# Autodesk Inventor assembly: 3 dubbele lagerblok assemble
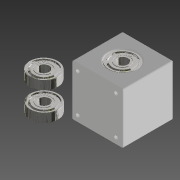
[picture p0: Inventor's stored thumbnail of the model, 180x180]
Saved by Autodesk Inventor 2020 (Build 240168000, 168)
## iProperties
Created: 2020-05-19
Part Number: 3 dubbele lagerblok assemble
Document SubType Name: Assembly
Designer: stefa
Author: stefa
## Documents named in this file (3)
- D:\github_gedeeld\BeerMinder\3D-model\axis5_6\3 dubbele lagerblok assemble.iam
- D:\github_gedeeld\BeerMinder\3D-model\axis5_6\3 dubbele lagerblok.ipt
- D:\github_gedeeld\BeerMinder\3D-model\bearings\Ball Bearing 608ZZ.ipt
## Components (4 placed, 2 different names)
1. 3 dubbele lagerblok:1 — Mate:1, Flush:1
2. Ball Bearing 608ZZ:1
3. Ball Bearing 608ZZ:2
4. Ball Bearing 608ZZ:3 — Mate:1, Flush:1
## Relationships (2: Mate 1, Flush 1)
- Mate:1: 3 dubbele lagerblok:1 ↔ Ball Bearing 608ZZ:3
- Flush:1 (0.5 mm): 3 dubbele lagerblok:1 ↔ Ball Bearing 608ZZ:3
